# Autodesk Inventor assembly: Ball Valve Assembly
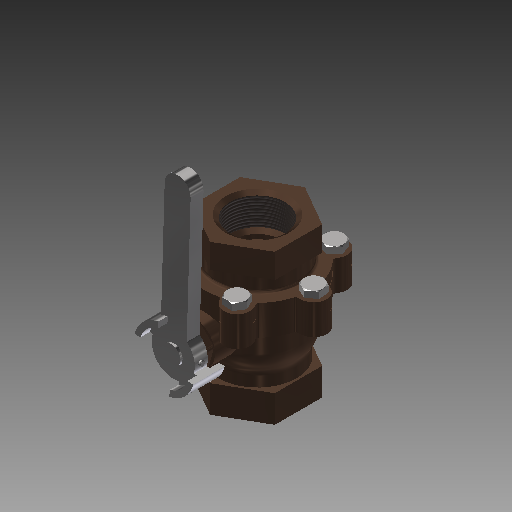
[picture p0: Inventor's stored thumbnail of the model, 512x512]
Saved by Autodesk Inventor 2018 (Build 220112000, 112)
## iProperties
Created: 2017-10-19
Part Number: Ball Valve Assembly
Document SubType Name: Assembly
Designer: kurtis
Author: kurtis
## Documents named in this file (10)
- D:\Users\kurti\Git-Home\CAD\GE101\MA6\Ball Valve Assembly.iam
- D:\Users\kurti\Git-Home\CAD\GE101\MA6\Bumper.ipt
- D:\Users\kurti\Git-Home\CAD\GE101\MA6\Handle.ipt
- D:\Users\kurti\Git-Home\CAD\GE101\MA6\Packing Nut Subassembly.iam
- D:\Users\kurti\Git-Home\CAD\GE101\MA6\Pin.ipt
- D:\Users\kurti\Git-Home\CAD\GE101\MA6\Stem.ipt
- D:\Users\kurti\Git-Home\CAD\GE101\MA6\Ball.ipt
- D:\Users\kurti\Git-Home\CAD\GE101\MA6\Body Cap Subassembly.iam
- D:\Users\kurti\Git-Home\CAD\GE101\MA6\Body.ipt
- D:\Users\kurti\Documents\Inventor\Content Center Files\R2018\en-US\ISO 4017(1)\ISO 4017 - M8 x 25 - ISO.ipt
## Components (14 placed, 9 different names)
1. Bumper:1 — Mate:4, Mate:5
2. Handle:1 — Cylindrical:2, Cylindrical:3
3. Packing Nut Subassembly:1 [sub-assembly] — Cylindrical:1, Cylindrical:4, Mate:3
4. Pin:1 — Rotational:1, Cylindrical:2
5. Stem:1 — Cylindrical:1, Rotational:1, Cylindrical:3, Planar:1, Mate:2
6. Ball:1 — Planar:1, Mate:1, Mate:2
7. Body Cap Subassembly:1 [sub-assembly] — Rotational:2, Rotational:3, Rotational:7, Rotational:6, Rotational:5, Rotational:4, Rotational:8, Rotational:9
8. Body:1 — Cylindrical:4, Mate:1, Mate:3, Mate:4, Mate:5, Rotational:2, Rotational:3
9. ISO 4017 M8 x 25:1 — Rotational:6
10. ISO 4017 M8 x 25:2 — Rotational:4
11. ISO 4017 M8 x 25:3 — Rotational:8
12. ISO 4017 M8 x 25:4 — Rotational:9
13. ISO 4017 M8 x 25:5 — Rotational:5
14. ISO 4017 M8 x 25:6 — Rotational:7
## Relationships (19: RevoluteJoint 9, Mate 5, CylindricalJoint 4, PlanarJoint 1)
- Cylindrical:1: Packing Nut Subassembly:1 ↔ Stem:1
- Rotational:1 [RevoluteJoint]: Pin:1 ↔ Stem:1
- Cylindrical:2: Handle:1 ↔ Pin:1
- Cylindrical:3: Handle:1 ↔ Stem:1
- Cylindrical:4: Packing Nut Subassembly:1 ↔ Body:1
- Planar:1: Stem:1 ↔ Ball:1
- Mate:1: Ball:1 ↔ Body:1
- Mate:2: Stem:1 ↔ Ball:1
- Mate:3: Packing Nut Subassembly:1 ↔ Body:1
- Mate:4: Bumper:1 ↔ Body:1
- Mate:5: Bumper:1 ↔ Body:1
- Rotational:2 [RevoluteJoint]: Body Cap Subassembly:1 ↔ Body:1
- Rotational:3 [RevoluteJoint]: Body Cap Subassembly:1 ↔ Body:1
- Rotational:7 [RevoluteJoint]: Body Cap Subassembly:1 ↔ ISO 4017 M8 x 25:6
- Rotational:6 [RevoluteJoint]: Body Cap Subassembly:1 ↔ ISO 4017 M8 x 25:1
- Rotational:5 [RevoluteJoint]: Body Cap Subassembly:1 ↔ ISO 4017 M8 x 25:5
- Rotational:4 [RevoluteJoint]: Body Cap Subassembly:1 ↔ ISO 4017 M8 x 25:2
- Rotational:8 [RevoluteJoint]: Body Cap Subassembly:1 ↔ ISO 4017 M8 x 25:3
- Rotational:9 [RevoluteJoint]: Body Cap Subassembly:1 ↔ ISO 4017 M8 x 25:4
